# Autodesk Inventor assembly: ESP Carillonneur 1
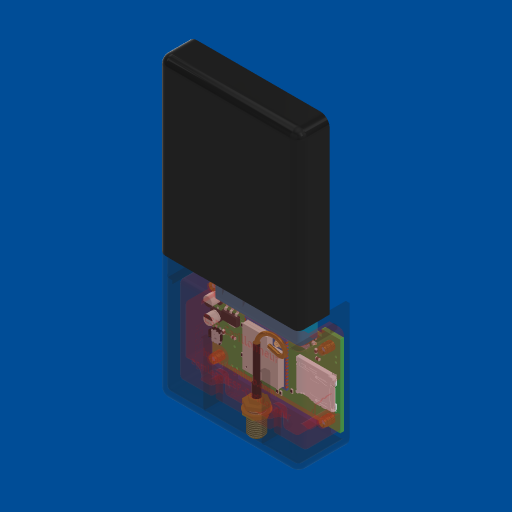
[picture p0: Inventor's stored thumbnail of the model, 512x512]
Saved by Autodesk Inventor 2023.2 (Build 272271000, 271)
## iProperties
Company: Kicad
Created: 2023-01-27
Part Number: ESP Carillonneur 1
Description: KiCad electronic assembly
Document SubType Name: Assembly
Designer: agmlego
Authority: Unknown
Mass: 57.2322 g
Surface Area: 841.267 cm^2
Volume: 68.8782 cm^3
Density: 0.83092 g/cm^3
Sending System: KiCad to STEP converter
Preprocessor: Open CASCADE STEP processor 7.6
Title: ESP Carillonneur.step
Author: Pcbnew
## Documents named in this file (20)
- D:\documents\projects\ESP Carillonneur\Mechanical CAD\ESP Carillonneur\ESP Carillonneur.iam
- D:\documents\projects\ESP Carillonneur\Mechanical CAD\R_0603_1608Metric.iam
- D:\documents\projects\ESP Carillonneur\Mechanical CAD\LED_0603_1608Metric.iam
- D:\documents\projects\ESP Carillonneur\Mechanical CAD\C_0603_1608Metric.iam
- D:\documents\projects\ESP Carillonneur\Mechanical CAD\SOT-223.iam
- D:\documents\projects\ESP Carillonneur\Mechanical CAD\ESP32-WROOM-32U.iam
- D:\documents\projects\ESP Carillonneur\Mechanical CAD\CP_Elec_4x4.5.iam
- D:\documents\projects\ESP Carillonneur\Mechanical CAD\_autosave-ESP Carillonneur PCB.ipt
- D:\documents\projects\ESP Carillonneur\Mechanical CAD\DM3AT-SF-PEJM5\DM3AT-SF-PEJM5.ipt
- D:\documents\projects\ESP Carillonneur\Mechanical CAD\EVQPU-LC-02K\EVQPU-LC-02K.ipt
- D:\documents\projects\ESP Carillonneur\Mechanical CAD\EEC12DRAN.ipt
- D:\documents\projects\ESP Carillonneur\Mechanical CAD\case.ipt
- D:\documents\projects\CreekFleet\CreekFleet_AutoBuoy\Mechanical CAD\hardware\94459A120_BRASS HEAT-SET INSERT FOR PLASTIC.ipt
- D:\documents\Inventor\Content Center Files\R2023\en-US\ANSI B18.3.1M(6)\ANSI B18.3.1M - M2x0.4 x 5(1).ipt
- D:\documents\projects\ESP Carillonneur\Mechanical CAD\rp-sma_pigtail.ipt
- D:\documents\projects\ESP Carillonneur\Mechanical CAD\rp-sma_washer.ipt
- D:\documents\projects\ESP Carillonneur\Mechanical CAD\rp-sma_nut.ipt
- D:\documents\projects\ESP Carillonneur\Mechanical CAD\AUS-200\sliding_door.ipt
- D:\documents\projects\ESP Carillonneur\Mechanical CAD\AUS-200\aus-200_top.ipt
- D:\documents\projects\ESP Carillonneur\Mechanical CAD\AUS-200\aus-200_bottom.ipt
## Components (37 placed, 31 different names)
1. rp-sma_nut:1 — Insert:13
2. rp-sma_washer:1 — Insert:12, Insert:13
3. rp-sma_pigtail:1 — Insert:11, Mate:8
4. 2 [sub-assembly]
5. 4 [sub-assembly]
6. 5 [sub-assembly]
7. 6 [sub-assembly]
8. 7 [sub-assembly]
9. 9 [sub-assembly]
10. 10 [sub-assembly]
11. 12 [sub-assembly]
12. 13 [sub-assembly]
13. 14 [sub-assembly]
14. 15 [sub-assembly]
15. 16 [sub-assembly]
16. 18 [sub-assembly]
17. 20 [sub-assembly]
18. 21 [sub-assembly]
19. 22 [sub-assembly]
20. 23 [sub-assembly]
21. 24 [sub-assembly]
22. 25 — Mate:1, Mate:2, Mate:3, Mate:4, Mate:5, Flush:1, Mate:6, Mate:7, Angle:1, Insert:5, Insert:6, Insert:7, Insert:8, Insert:9, Insert:10
23. DM3AT-SF-PEJM5:1 — Mate:1, Mate:5, Flush:1
24. EVQPU-LC-02K:1 — Mate:2, Mate:3, Mate:4
25. EEC12DRAN:1 — Mate:6, Mate:7, Angle:1, Mate:9
26. case:1 — Insert:1, Insert:2, Insert:3, Insert:4, Insert:11, Mate:8, Insert:12, Flush:2, Mate:10
27. 94459A120_BRASS HEAT-SET INSERT FOR PLASTIC:1 — Insert:2
28. 94459A120_BRASS HEAT-SET INSERT FOR PLASTIC:2 — Insert:3
29. 94459A120_BRASS HEAT-SET INSERT FOR PLASTIC:3 — Insert:4, Insert:6
30. 94459A120_BRASS HEAT-SET INSERT FOR PLASTIC:4 — Insert:1, Insert:5
31. Forged Socket Head Cap Screw - Metric M2x0.4 x 5:1 — Insert:7
32. Forged Socket Head Cap Screw - Metric M2x0.4 x 5:2 — Insert:8
33. Forged Socket Head Cap Screw - Metric M2x0.4 x 5:3 — Insert:9
34. Forged Socket Head Cap Screw - Metric M2x0.4 x 5:4 — Insert:10
35. sliding_door:1 — Insert:14, Insert:15
36. aus-200_top:1 — Insert:14, Insert:15, Insert:16, Insert:17
37. aus-200_bottom:1 — Insert:16, Insert:17, Flush:2, Mate:9, Mate:10
## Relationships (30: Insert 17, Mate 10, Flush 2, Angle 1)
- Mate:1: 25 ↔ DM3AT-SF-PEJM5:1
- Mate:2: 25 ↔ EVQPU-LC-02K:1
- Mate:3: 25 ↔ EVQPU-LC-02K:1
- Mate:4: 25 ↔ EVQPU-LC-02K:1
- Mate:5 (3.313 mm): 25 ↔ DM3AT-SF-PEJM5:1
- Flush:1 (1.341 mm): 25 ↔ DM3AT-SF-PEJM5:1
- Mate:6: 25 ↔ EEC12DRAN:1
- Mate:7: 25 ↔ EEC12DRAN:1
- Angle:1 (180 deg): 25 ↔ EEC12DRAN:1
- Insert:1: case:1 ↔ 94459A120_BRASS HEAT-SET INSERT FOR PLASTIC:4
- Insert:2: case:1 ↔ 94459A120_BRASS HEAT-SET INSERT FOR PLASTIC:1
- Insert:3: case:1 ↔ 94459A120_BRASS HEAT-SET INSERT FOR PLASTIC:2
- Insert:4: case:1 ↔ 94459A120_BRASS HEAT-SET INSERT FOR PLASTIC:3
- Insert:5: 25 ↔ 94459A120_BRASS HEAT-SET INSERT FOR PLASTIC:4
- Insert:6: 25 ↔ 94459A120_BRASS HEAT-SET INSERT FOR PLASTIC:3
- Insert:7: 25 ↔ Forged Socket Head Cap Screw - Metric M2x0.4 x 5:1
- Insert:8: 25 ↔ Forged Socket Head Cap Screw - Metric M2x0.4 x 5:2
- Insert:9: 25 ↔ Forged Socket Head Cap Screw - Metric M2x0.4 x 5:3
- Insert:10: 25 ↔ Forged Socket Head Cap Screw - Metric M2x0.4 x 5:4
- Insert:11: rp-sma_pigtail:1 ↔ case:1
- Mate:8: rp-sma_pigtail:1 ↔ case:1
- Insert:12: rp-sma_washer:1 ↔ case:1
- Insert:13: rp-sma_nut:1 ↔ rp-sma_washer:1
- Insert:14: sliding_door:1 ↔ aus-200_top:1
- Insert:15: sliding_door:1 ↔ aus-200_top:1
- Insert:16: aus-200_top:1 ↔ aus-200_bottom:1
- Insert:17: aus-200_top:1 ↔ aus-200_bottom:1
- Flush:2: case:1 ↔ aus-200_bottom:1
- Mate:9 (1.2025 mm): EEC12DRAN:1 ↔ aus-200_bottom:1
- Mate:10 (11 mm): case:1 ↔ aus-200_bottom:1
